# Autodesk Inventor assembly: FullV2
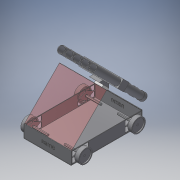
[picture p0: Inventor's stored thumbnail of the model, 180x180]
Saved by Autodesk Inventor 2019 (Build 230136000, 136)
## iProperties
Created: 2021-09-16
Part Number: FullV2
Document SubType Name: Assembly
Designer: timmy
Author: timmy
## Documents named in this file (11)
- S:\Inventor\RoboCatz\T-Shirt\FullV2.iam
- S:\Inventor\RoboCatz\T-Shirt\NamePlateV1.ipt
- S:\Inventor\RoboCatz\T-Shirt\R-O-SideV1.ipt
- S:\Inventor\RoboCatz\T-Shirt\TopV2.ipt
- S:\Inventor\RoboCatz\T-Shirt\Plexi-SideV!.ipt
- S:\Inventor\RoboCatz\T-Shirt\BackV1.ipt
- S:\Inventor\RoboCatz\T-Shirt\LauncherFullV1.iam
- S:\Inventor\RoboCatz\T-Shirt\BottomV1.ipt
- S:\Inventor\RoboCatz\T-Shirt\AxleBearingV1.ipt
- S:\Inventor\RoboCatz\T-Shirt\6x10inAxleV1.ipt
- S:\Inventor\RoboCatz\T-Shirt\WheelV1.ipt
## Components (22 placed, 10 different names)
1. NamePlateV1:1 — Mate:1, Flush:2, Flush:3, Flush:4, Flush:5, Flush:6, Flush:14
2. R-O-SideV1:1 — Flush:4, Flush:5, Flush:6, Mate:6, Flush:11, Mate:9, Mate:10, Mate:30, Mate:31, Mate:36, Mate:37
3. NamePlateV1:2 — Flush:7, Flush:8, Flush:9
4. R-O-SideV1:2 — Mate:1, Flush:2, Flush:3, Flush:7, Flush:8, Flush:9, Mate:2, Angle:1, Mate:3, Angle:3, Flush:10, Mate:7, Mate:8, Mate:17, Flush:15, Mate:18, Mate:19, Mate:24, Mate:25, Angle:4
5. Plexi-SideV!:1 — Flush:11, Mate:9, Mate:10, Mate:12
6. Plexi-SideV!:2 — Flush:10, Mate:7, Mate:8, Mate:11, Flush:12, Flush:13
7. TopV2:1 — Mate:11, Flush:12, Mate:13
8. BackV1:1 — Mate:12, Mate:13, Flush:13, Mate:14, Mate:15, Mate:16
9. LauncherFullV1:1 [sub-assembly] — Mate:14, Mate:15, Mate:16
10. BottomV1:1 — Flush:14, Mate:17, Flush:15
11. AxleBearingV1:1 — Mate:30, Mate:31, Flush:20, Mate:32, Mate:33
12. AxleBearingV1:2 — Mate:36, Mate:37, Flush:36, Mate:38, Mate:39
13. AxleBearingV1:3 — Mate:24, Mate:25, Flush:18, Mate:26, Mate:27
14. AxleBearingV1:4 — Mate:18, Mate:19, Mate:20, Flush:16, Mate:21
15. 6x10inAxleV1:1 — Mate:20, Flush:16, Mate:21, Flush:17, Mate:22, Mate:23
16. WheelV1:1 — Flush:17, Mate:22, Mate:23
17. WheelV1:2 — Flush:41, Mate:41, Mate:42
18. WheelV1:3 — Flush:19, Mate:28, Mate:29
19. WheelV1:4 — Flush:35, Mate:34, Mate:35
20. 6x10inAxleV1:2 — Flush:36, Mate:38, Mate:39, Flush:41, Mate:41, Mate:42, Flush:42
21. 6x10inAxleV1:3 — Flush:20, Mate:32, Mate:33, Flush:35, Mate:34, Mate:35
22. 6x10inAxleV1:4 — Flush:18, Mate:26, Mate:27, Flush:19, Mate:28, Mate:29, Flush:42, Angle:4
## Relationships (66: Mate 39, Flush 23, Angle 4)
- Mate:1: NamePlateV1:1 ↔ R-O-SideV1:2
- Flush:2: NamePlateV1:1 ↔ R-O-SideV1:2
- Flush:3: NamePlateV1:1 ↔ R-O-SideV1:2
- Flush:4: NamePlateV1:1 ↔ R-O-SideV1:1
- Flush:5: NamePlateV1:1 ↔ R-O-SideV1:1
- Flush:6: NamePlateV1:1 ↔ R-O-SideV1:1
- Flush:7: NamePlateV1:2 ↔ R-O-SideV1:2
- Flush:8: NamePlateV1:2 ↔ R-O-SideV1:2
- Flush:9: NamePlateV1:2 ↔ R-O-SideV1:2
- Mate:2: R-O-SideV1:2
- Angle:1 (45 deg): R-O-SideV1:2
- Mate:3: R-O-SideV1:2
- Angle:2 (90 deg)
- Mate:6: R-O-SideV1:1
- Angle:3 (135 deg): R-O-SideV1:2
- Flush:10: R-O-SideV1:2 ↔ Plexi-SideV!:2
- Mate:7: R-O-SideV1:2 ↔ Plexi-SideV!:2
- Mate:8: R-O-SideV1:2 ↔ Plexi-SideV!:2
- Flush:11: R-O-SideV1:1 ↔ Plexi-SideV!:1
- Mate:9: R-O-SideV1:1 ↔ Plexi-SideV!:1
- Mate:10: R-O-SideV1:1 ↔ Plexi-SideV!:1
- Mate:11: Plexi-SideV!:2 ↔ TopV2:1
- Flush:12: Plexi-SideV!:2 ↔ TopV2:1
- Mate:12: Plexi-SideV!:1 ↔ BackV1:1
- Mate:13: TopV2:1 ↔ BackV1:1
- Flush:13: Plexi-SideV!:2 ↔ BackV1:1
- Mate:14: BackV1:1 ↔ LauncherFullV1:1
- Mate:15: BackV1:1 ↔ LauncherFullV1:1
- Mate:16: BackV1:1 ↔ LauncherFullV1:1
- Flush:14: NamePlateV1:1 ↔ BottomV1:1
- Mate:17: R-O-SideV1:2 ↔ BottomV1:1
- Flush:15: R-O-SideV1:2 ↔ BottomV1:1
- Mate:18: R-O-SideV1:2 ↔ AxleBearingV1:4
- Mate:19: R-O-SideV1:2 ↔ AxleBearingV1:4
- Mate:20: AxleBearingV1:4 ↔ 6x10inAxleV1:1
- Flush:16 (50.8 mm): AxleBearingV1:4 ↔ 6x10inAxleV1:1
- Mate:21: AxleBearingV1:4 ↔ 6x10inAxleV1:1
- Flush:17: 6x10inAxleV1:1 ↔ WheelV1:1
- Mate:22: 6x10inAxleV1:1 ↔ WheelV1:1
- Mate:23: 6x10inAxleV1:1 ↔ WheelV1:1
- Mate:24: R-O-SideV1:2 ↔ AxleBearingV1:3
- Mate:25: R-O-SideV1:2 ↔ AxleBearingV1:3
- Flush:18 (50.8 mm): AxleBearingV1:3 ↔ 6x10inAxleV1:4
- Mate:26: AxleBearingV1:3 ↔ 6x10inAxleV1:4
- Mate:27: AxleBearingV1:3 ↔ 6x10inAxleV1:4
- Flush:19: WheelV1:3 ↔ 6x10inAxleV1:4
- Mate:28: WheelV1:3 ↔ 6x10inAxleV1:4
- Mate:29: WheelV1:3 ↔ 6x10inAxleV1:4
- Mate:30: R-O-SideV1:1 ↔ AxleBearingV1:1
- Mate:31: R-O-SideV1:1 ↔ AxleBearingV1:1
- Flush:20 (50.8 mm): AxleBearingV1:1 ↔ 6x10inAxleV1:3
- Mate:32: AxleBearingV1:1 ↔ 6x10inAxleV1:3
- Mate:33: AxleBearingV1:1 ↔ 6x10inAxleV1:3
- Flush:35: WheelV1:4 ↔ 6x10inAxleV1:3
- Mate:34: WheelV1:4 ↔ 6x10inAxleV1:3
- Mate:35: WheelV1:4 ↔ 6x10inAxleV1:3
- Mate:36: R-O-SideV1:1 ↔ AxleBearingV1:2
- Mate:37: R-O-SideV1:1 ↔ AxleBearingV1:2
- Flush:36 (-50.8 mm): AxleBearingV1:2 ↔ 6x10inAxleV1:2
- Mate:38: AxleBearingV1:2 ↔ 6x10inAxleV1:2
- Mate:39: AxleBearingV1:2 ↔ 6x10inAxleV1:2
- Flush:41: WheelV1:2 ↔ 6x10inAxleV1:2
- Mate:41: WheelV1:2 ↔ 6x10inAxleV1:2
- Mate:42: WheelV1:2 ↔ 6x10inAxleV1:2
- Flush:42: 6x10inAxleV1:2 ↔ 6x10inAxleV1:4
- Angle:4 (0 deg): R-O-SideV1:2 ↔ 6x10inAxleV1:4
